# Autodesk Inventor assembly: ForkMountWithCelestronTubeConnector
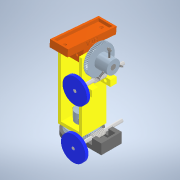
[picture p0: Inventor's stored thumbnail of the model, 180x180]
Saved by Autodesk Inventor 2021.1 (Build 251245010, 245A)
## iProperties
Created: 2020-07-21
Part Number: ForkMountWithCelestronTubeConnector
Document SubType Name: Assembly
Designer: robst
Mass: 6586.24 g
Surface Area: 6637.23 cm^2
Volume: 2932.35 cm^3
Density: 2.24606 g/cm^3
Author: robst
## Documents named in this file (13)
- C:\git\CAD-Development\robSteele\ShapeWays\TelescopeProjects\TelescopeMount\ForkMountWithCelestronTubeConnector.iam
- C:\git\CAD-Development\robSteele\ShapeWays\TelescopeProjects\TelescopeMount\forkV02.ipt
- C:\git\CAD-Development\robSteele\ShapeWays\TelescopeProjects\TelescopeMount\celestronTubeBracket.ipt
- C:\git\CAD-Development\robSteele\ShapeWays\TelescopeProjects\TelescopeMount\telescopeTube.ipt
- C:\git\CAD-Development\robSteele\ShapeWays\TelescopeProjects\TelescopeMount\connectorToTubeBrackets03.ipt
- C:\git\CAD-Development\robSteele\ShapeWays\TelescopeProjects\TelescopeMount\ForkMountWithCelestronTubeConnector\Design Accelerator\Worm Gears2.iam
- C:\git\CAD-Development\robSteele\ShapeWays\TelescopeProjects\TelescopeMount\celestronMountDecHandleAssembly.iam
- C:\git\CAD-Development\robSteele\ShapeWays\TelescopeProjects\TelescopeMount\steeleAxel-0_625.ipt
- C:\git\CAD-Development\robSteele\ShapeWays\TelescopeProjects\TelescopeMount\celestronTripodAdapterAssembly.iam
- C:\git\CAD-Development\robSteele\ShapeWays\TelescopeProjects\TelescopeMount\6x3_8-keyedDriveShaft.ipt
- c:\git\CAD-MfgResources\McMaster-Carr\Insert\10-32x0_375-94459A360_BRASS HEAT-SET INSERT FOR PLASTIC.ipt
- C:\Users\robst\Documents\Inventor\Content Center Files\R2021\en-US\ANSI B18.17(29)\ANSI B18.17 - 10-32 UNF - 1B (12).ipt
- C:\Users\robst\Documents\Inventor\Content Center Files\R2021\en-US\ANSI B18.17(29)\ANSI B18.17 - 10-32 UNF - 0.75B (12).ipt
## Components (27 placed, 12 different names)
1. forkV02:1 — Insert:3, Mate:6, Flush:3, Insert:8, Mate:7
2. celestronTubeBracket:1 — Insert:2, Mate:3, Mate:4
3. connectorToTubeBrackets03:1 — Mate:1, Mate:2, Mate:3, Mate:4, Insert:3
4. celestronTubeBracket:2 — Mate:1, Mate:2
5. telescopeTube:1 — Insert:2
6. Worm Gears:1 [sub-assembly] — Mate:6, Flush:3, Insert:4, Insert:7, Insert:13, Mate:7
7. 6x3_8-keyedDriveShaft:1 — Insert:4, Insert:5, Insert:6
8. celestronMountDecHandleAssembly:1 [sub-assembly] — Insert:5
9. celestronMountDecHandleAssembly:2 [sub-assembly] — Insert:6
10. celestronTripodAdapterAssembly:1 [sub-assembly] — Insert:9
11. steeleAxel-0_625:1 — Insert:7
12. Worm Gears:2 [sub-assembly] — Insert:8, Insert:9, Insert:10, Insert:15
13. 6x3_8-keyedDriveShaft:2 — Insert:10, Insert:11, Insert:12
14. celestronMountDecHandleAssembly:3 [sub-assembly] — Insert:11
15. celestronMountDecHandleAssembly:4 [sub-assembly] — Insert:12
16. 10-32x0_375-94459A360_BRASS HEAT-SET INSERT FOR PLASTIC:1 — Insert:13, Insert:14
17. 10-32x0_375-94459A360_BRASS HEAT-SET INSERT FOR PLASTIC:2
18. 10-32x0_375-94459A360_BRASS HEAT-SET INSERT FOR PLASTIC:3
19. Type B - Regular Thumb Screw - Plain Point - Inch 10-32 UNF - 1:1 — Insert:14
20. Type B - Regular Thumb Screw - Plain Point - Inch 10-32 UNF - 1:2
21. Type B - Regular Thumb Screw - Plain Point - Inch 10-32 UNF - 1:3
22. 10-32x0_375-94459A360_BRASS HEAT-SET INSERT FOR PLASTIC:4 — Insert:15, Insert:16
23. Type B - Regular Thumb Screw - Plain Point - Inch 10-32 UNF - 0.75:1 — Insert:16
24. 10-32x0_375-94459A360_BRASS HEAT-SET INSERT FOR PLASTIC:5
25. Type B - Regular Thumb Screw - Plain Point - Inch 10-32 UNF - 0.75:2
26. 10-32x0_375-94459A360_BRASS HEAT-SET INSERT FOR PLASTIC:6
27. Type B - Regular Thumb Screw - Plain Point - Inch 10-32 UNF - 0.75:3
## Component patterns: (3 elements, first: 10-32x0_375-94459A360_BRASS HEAT-SET INSERT FOR PLASTIC:1), (3 elements, first: Type B - Regular Thumb Screw - Plain Point - Inch 10-32 UNF - 1:1), (3 elements, first: 10-32x0_375-94459A360_BRASS HEAT-SET INSERT FOR PLASTIC:4 + Type B - Regular Thumb Screw - Plain Point - Inch 10-32 UNF - 0.75:1)
## Relationships (24: Insert 15, Mate 6, Flush 3)
- [Flush]: celestronTubeBracket:1 ↔ connectorToTubeBrackets03:1
- [Flush]: connectorToTubeBrackets03:1 ↔ celestronTubeBracket:2
- Insert:2 (-330.2 mm): celestronTubeBracket:1 ↔ telescopeTube:1
- Mate:1: connectorToTubeBrackets03:1 ↔ celestronTubeBracket:2
- Mate:2: connectorToTubeBrackets03:1 ↔ celestronTubeBracket:2
- Mate:3: celestronTubeBracket:1 ↔ connectorToTubeBrackets03:1
- Mate:4: celestronTubeBracket:1 ↔ connectorToTubeBrackets03:1
- Insert:3: forkV02:1 ↔ connectorToTubeBrackets03:1
- Mate:6 (9.525 mm): forkV02:1 ↔ Worm Gears:1
- Flush:3: forkV02:1 ↔ Worm Gears:1
- Insert:4 (57.15 mm): Worm Gears:1 ↔ 6x3_8-keyedDriveShaft:1
- Insert:5: 6x3_8-keyedDriveShaft:1 ↔ celestronMountDecHandleAssembly:1
- Insert:6: 6x3_8-keyedDriveShaft:1 ↔ celestronMountDecHandleAssembly:2
- Insert:7: Worm Gears:1 ↔ steeleAxel-0_625:1
- Insert:8: forkV02:1 ↔ Worm Gears:2
- Insert:9: celestronTripodAdapterAssembly:1 ↔ Worm Gears:2
- Insert:10 (-57.15 mm): Worm Gears:2 ↔ 6x3_8-keyedDriveShaft:2
- Insert:11: 6x3_8-keyedDriveShaft:2 ↔ celestronMountDecHandleAssembly:3
- Insert:12: 6x3_8-keyedDriveShaft:2 ↔ celestronMountDecHandleAssembly:4
- Insert:13: Worm Gears:1 ↔ 10-32x0_375-94459A360_BRASS HEAT-SET INSERT FOR PLASTIC:1
- Insert:14: 10-32x0_375-94459A360_BRASS HEAT-SET INSERT FOR PLASTIC:1 ↔ Type B - Regular Thumb Screw - Plain Point - Inch 10-32 UNF - 1:1
- Insert:15: Worm Gears:2 ↔ 10-32x0_375-94459A360_BRASS HEAT-SET INSERT FOR PLASTIC:4
- Insert:16 (-12.7 mm): 10-32x0_375-94459A360_BRASS HEAT-SET INSERT FOR PLASTIC:4 ↔ Type B - Regular Thumb Screw - Plain Point - Inch 10-32 UNF - 0.75:1
- Mate:7: forkV02:1 ↔ Worm Gears:1
